# Autodesk Inventor assembly: HbArduinoMicroShield01
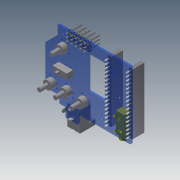
[picture p0: Inventor's stored thumbnail of the model, 180x180]
Saved by Autodesk Inventor 2015 SP1 (Build 190203100, 203)
## iProperties
Created: 2015-02-16
Part Number: HbArduinoMicroShield01
Document SubType Name: Assembly
Designer: Yamaura
Author: Yamaura
## Documents named in this file (8)
- C:\Users\Yamaura\Documents\GitHub\HACKberry\HACKberry-hardware\3D\Inventor\Parts\HbArduinoMicroShield01.iam
- C:\Users\Yamaura\Documents\GitHub\HACKberry\HACKberry-hardware\3D\Inventor\Parts\ArduinoMicroShieldBoard01.ipt
- C:\Users\Yamaura\Documents\GitHub\HACKberry\HACKberry-hardware\3D\Inventor\Parts\PinSocketU01.iam
- C:\Users\Yamaura\Documents\GitHub\HACKberry\HACKberry-hardware\3D\Inventor\Parts\pin_header_3 Pin.ipt
- C:\Users\Yamaura\Documents\GitHub\HACKberry\HACKberry-hardware\3D\Inventor\Parts\MJ179PH.ipt
- C:\Users\Yamaura\Documents\GitHub\HACKberry\HACKberry-hardware\3D\Inventor\Parts\SKRGAQD010.ipt
- C:\Users\Yamaura\Documents\GitHub\HACKberry\HACKberry-hardware\3D\Inventor\Parts\SS-12SDP2.ipt
- C:\Users\Yamaura\Documents\GitHub\HACKberry\HACKberry-hardware\3D\Inventor\Parts\MJ-4535-3.ipt
## Components (47 placed, 7 different names)
1. ArduinoMicroShieldBoard01:1 — メイト:1, メイト:2, メイト:5, メイト:8, 角度:3, フラッシュ:10, フラッシュ:11, メイト:9, メイト:10, フラッシュ:12, メイト:12, メイト:13, メイト:14, メイト:15, メイト:16, メイト:17, メイト:18, メイト:19, メイト:20, メイト:21, メイト:22, メイト:23, メイト:26, メイト:27, メイト:28, メイト:29, メイト:30, メイト:31
2. MJ179PH:1 — メイト:10, フラッシュ:12, メイト:11
3. SKRGAQD010:1 — メイト:15, メイト:22, メイト:23
4. SKRGAQD010:2 — メイト:14, メイト:20, メイト:21
5. SKRGAQD010:3 — メイト:13, メイト:18, メイト:19
6. SKRGAQD010:4 — メイト:12, メイト:16, メイト:17
7. SS-12SDP2:1 — メイト:26, メイト:27, メイト:28
8. MJ-4535-3:1 — メイト:29, メイト:30, メイト:31
9. pin_header_3 Pin:1 — メイト:5, メイト:8, メイト:9
10. pin_header_3 Pin:2
11. pin_header_3 Pin:3
12. pin_header_3 Pin:4
13. pin_header_3 Pin:5
14. PinSocketU01:1 [sub-assembly] — メイト:1, メイト:2, 角度:1
15. PinSocketU01:2 [sub-assembly]
16. PinSocketU01:3 [sub-assembly]
17. PinSocketU01:4 [sub-assembly]
18. PinSocketU01:5 [sub-assembly]
19. PinSocketU01:6 [sub-assembly]
20. PinSocketU01:7 [sub-assembly]
21. PinSocketU01:8 [sub-assembly]
22. PinSocketU01:9 [sub-assembly]
23. PinSocketU01:10 [sub-assembly]
24. PinSocketU01:11 [sub-assembly]
25. PinSocketU01:12 [sub-assembly]
26. PinSocketU01:13 [sub-assembly]
27. PinSocketU01:14 [sub-assembly]
28. PinSocketU01:15 [sub-assembly]
29. PinSocketU01:16 [sub-assembly]
30. PinSocketU01:17 [sub-assembly]
31. PinSocketU01:18 [sub-assembly]
32. PinSocketU01:19 [sub-assembly]
33. PinSocketU01:20 [sub-assembly]
34. PinSocketU01:21 [sub-assembly]
35. PinSocketU01:22 [sub-assembly]
36. PinSocketU01:23 [sub-assembly]
37. PinSocketU01:24 [sub-assembly]
38. PinSocketU01:25 [sub-assembly]
39. PinSocketU01:26 [sub-assembly]
40. PinSocketU01:27 [sub-assembly]
41. PinSocketU01:28 [sub-assembly]
42. PinSocketU01:29 [sub-assembly]
43. PinSocketU01:30 [sub-assembly]
44. PinSocketU01:31 [sub-assembly]
45. PinSocketU01:32 [sub-assembly]
46. PinSocketU01:33 [sub-assembly]
47. PinSocketU01:34 [sub-assembly]
## Component patterns: (2 elements), (5 elements, first: pin_header_3 Pin:1), (17 elements, first: PinSocketU01:1), コンポーネント パターン 1:2 (17 elements)
## Relationships (30: Mate 25, Flush 3, Angle 2)
- メイト:1 [Mate]: ArduinoMicroShieldBoard01:1 ↔ PinSocketU01:1
- メイト:2 [Mate]: ArduinoMicroShieldBoard01:1 ↔ PinSocketU01:1
- 角度:1 [Angle] (0 deg): PinSocketU01:1
- メイト:5 [Mate]: ArduinoMicroShieldBoard01:1 ↔ pin_header_3 Pin:1
- メイト:8 [Mate]: ArduinoMicroShieldBoard01:1 ↔ pin_header_3 Pin:1
- 角度:3 [Angle] (0 deg): ArduinoMicroShieldBoard01:1
- フラッシュ:10 [Flush]: ArduinoMicroShieldBoard01:1
- フラッシュ:11 [Flush]: ArduinoMicroShieldBoard01:1
- メイト:9 [Mate]: ArduinoMicroShieldBoard01:1 ↔ pin_header_3 Pin:1
- メイト:10 [Mate]: ArduinoMicroShieldBoard01:1 ↔ MJ179PH:1
- フラッシュ:12 [Flush]: ArduinoMicroShieldBoard01:1 ↔ MJ179PH:1
- メイト:11 [Mate] (-36.8 mm): MJ179PH:1
- メイト:12 [Mate]: ArduinoMicroShieldBoard01:1 ↔ SKRGAQD010:4
- メイト:13 [Mate]: ArduinoMicroShieldBoard01:1 ↔ SKRGAQD010:3
- メイト:14 [Mate]: ArduinoMicroShieldBoard01:1 ↔ SKRGAQD010:2
- メイト:15 [Mate]: ArduinoMicroShieldBoard01:1 ↔ SKRGAQD010:1
- メイト:16 [Mate]: ArduinoMicroShieldBoard01:1 ↔ SKRGAQD010:4
- メイト:17 [Mate]: ArduinoMicroShieldBoard01:1 ↔ SKRGAQD010:4
- メイト:18 [Mate]: ArduinoMicroShieldBoard01:1 ↔ SKRGAQD010:3
- メイト:19 [Mate]: ArduinoMicroShieldBoard01:1 ↔ SKRGAQD010:3
- メイト:20 [Mate]: ArduinoMicroShieldBoard01:1 ↔ SKRGAQD010:2
- メイト:21 [Mate]: ArduinoMicroShieldBoard01:1 ↔ SKRGAQD010:2
- メイト:22 [Mate]: ArduinoMicroShieldBoard01:1 ↔ SKRGAQD010:1
- メイト:23 [Mate]: ArduinoMicroShieldBoard01:1 ↔ SKRGAQD010:1
- メイト:26 [Mate]: ArduinoMicroShieldBoard01:1 ↔ SS-12SDP2:1
- メイト:27 [Mate]: ArduinoMicroShieldBoard01:1 ↔ SS-12SDP2:1
- メイト:28 [Mate]: ArduinoMicroShieldBoard01:1 ↔ SS-12SDP2:1
- メイト:29 [Mate]: ArduinoMicroShieldBoard01:1 ↔ MJ-4535-3:1
- メイト:30 [Mate]: ArduinoMicroShieldBoard01:1 ↔ MJ-4535-3:1
- メイト:31 [Mate]: ArduinoMicroShieldBoard01:1 ↔ MJ-4535-3:1
